# Autodesk Inventor assembly: corner pieces + screw
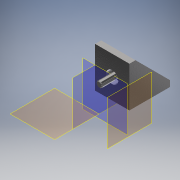
[picture p0: Inventor's stored thumbnail of the model, 180x180]
Saved by Autodesk Inventor 2017 (Build 210142000, 142)
## iProperties
Part Number: corner pieces + screw
Material: Generisch
Document SubType Name: Assembly
Designer: Till
Author: Till
## Documents named in this file (3)
- C:\Users\Till\Dropbox\DIY\CoreBot\corner pieces + screw.iam
- C:\Users\Till\Dropbox\DIY\CAD\Corner Piece.ipt
- C:\Users\Till\Dropbox\DIY\CoreBot\M3 x 10.ipt
## Components (3 placed, 2 different names)
1. Corner Piece:1 — Passend:1, Passend:2, Passend:3, Passend:4
2. M3 x 10:1 — Passend:2, Passend:3
3. M3 x 10:2 — Passend:1, Passend:4
## Relationships (4: Mate 4)
- Passend:1 [Mate]: Corner Piece:1 ↔ M3 x 10:2
- Passend:2 [Mate]: Corner Piece:1 ↔ M3 x 10:1
- Passend:3 [Mate]: Corner Piece:1 ↔ M3 x 10:1
- Passend:4 [Mate]: Corner Piece:1 ↔ M3 x 10:2
